# Autodesk Inventor assembly: pink-suspension
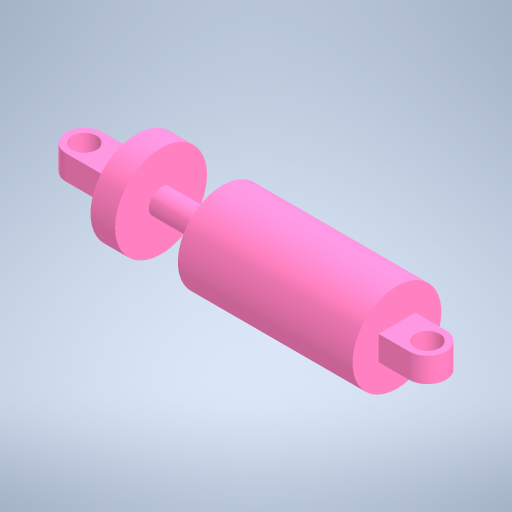
[picture p0: Inventor's stored thumbnail of the model, 512x512]
Saved by Autodesk Inventor 2024.1 (Build 281209000, 209)
## iProperties
Created: 2023-11-21
Part Number: pink-suspension
Document SubType Name: Assembly
Designer: haruy
Author: haruy
## Documents named in this file (3)
- C:\Users\haruy\OneDrive - Kyushu University\KURT_工房共有\2023~2024\ハード\CAD\2024NHK\000_parts\サスペンション\pink-suspension.iam
- C:\Users\haruy\OneDrive - Kyushu University\KURT_工房共有\2023~2024\ハード\CAD\2024NHK\000_parts\サスペンション\pink-suspension-top.ipt
- C:\Users\haruy\OneDrive - Kyushu University\KURT_工房共有\2023~2024\ハード\CAD\2024NHK\000_parts\サスペンション\pink-suspension-under.ipt
## Components (2 placed, 2 different names)
1. pink-suspension-top:1 — フラッシュ:1, 円柱状:1
2. pink-suspension-under:1 — フラッシュ:1, 円柱状:1
## Relationships (2: Flush 1, CylindricalJoint 1)
- フラッシュ:1 [Flush]: pink-suspension-top:1 ↔ pink-suspension-under:1
- 円柱状:1 [CylindricalJoint]: pink-suspension-top:1 ↔ pink-suspension-under:1
